# Autodesk Inventor assembly: MainAssembly
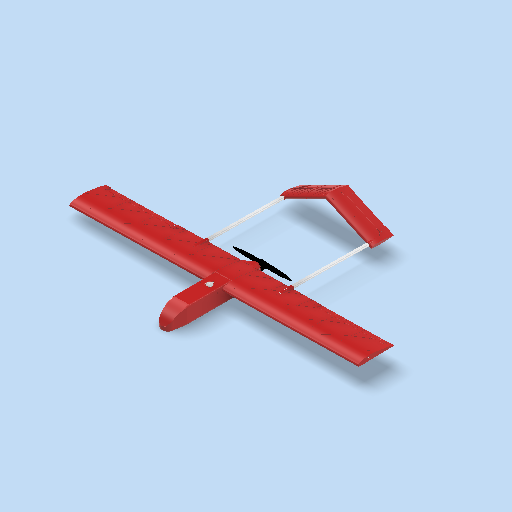
[picture p0: Inventor's stored thumbnail of the model, 512x512]
Saved by Autodesk Inventor 2026.1 (Build 301233000, 233)
## iProperties
Created: 2025-08-01
Part Number: MainAssembly
Document SubType Name: Assembly
Designer: Cupri
Author: Cupri
## Documents named in this file (29)
- C:\GitHub\SWIFT-UAV\System_development\Pelican\structural_model\v0.3.0\MainAssembly\MainAssembly.iam
- C:\GitHub\SWIFT-UAV\System_development\Pelican\structural_model\v0.3.0\Parts\WingParts\WingBox.ipt
- C:\GitHub\SWIFT-UAV\System_development\Pelican\structural_model\v0.3.0\Parts\WingParts\WingLeft_v0.1.ipt
- C:\GitHub\SWIFT-UAV\System_development\Pelican\structural_model\v0.3.0\Parts\Extrusion\20x20x1295ExtrudedAluminum.ipt
- C:\GitHub\SWIFT-UAV\System_development\Pelican\structural_model\v0.3.0\Parts\Extrusion\20x20x800ExtrudedAluminum.ipt
- C:\GitHub\SWIFT-UAV\System_development\Pelican\structural_model\v0.3.0\Parts\MotorHousing.ipt
- C:\GitHub\SWIFT-UAV\System_development\Pelican\structural_model\v0.3.0\Parts\Fueselage.ipt
- C:\GitHub\SWIFT-UAV\System_development\Pelican\structural_model\v0.3.0\Parts\FrontCover.ipt
- C:\GitHub\SWIFT-UAV\System_development\Pelican\structural_model\v0.3.0\Parts\AlerionLeft.ipt
- C:\GitHub\SWIFT-UAV\System_development\Pelican\structural_model\v0.3.0\Parts\Extrusion\20x20x1295ExtrudedAluminum_MIR.ipt
- C:\GitHub\SWIFT-UAV\System_development\Pelican\structural_model\v0.3.0\Parts\WingParts\WingLeft_v0.1_MIR1.ipt
- C:\GitHub\SWIFT-UAV\System_development\Pelican\structural_model\v0.3.0\Parts\Extrusion\20x20x800ExtrudedAluminum_MIR2.ipt
- C:\GitHub\SWIFT-UAV\System_development\Pelican\structural_model\v0.3.0\Parts\Vtail.ipt
- C:\GitHub\SWIFT-UAV\System_development\Pelican\structural_model\v0.3.0\Parts\Vtail_MIR.ipt
- C:\GitHub\SWIFT-UAV\System_development\Pelican\structural_model\v0.3.0\Parts\AlerionLeft_MIR1.ipt
- C:\GitHub\SWIFT-UAV\System_development\Pelican\structural_model\v0.3.0\Parts\Extrusion\20x20x785ExtrudedAluminum.ipt
- C:\GitHub\SWIFT-UAV\System_development\Pelican\structural_model\v0.3.0\Parts\Mount v2.ipt
- C:\GitHub\SWIFT-UAV\System_development\Pelican\structural_model\v0.3.0\Parts\kst-ds215mg-servo-1.snapshot.4\KST_DS215MG\KST_DS215MG\KST_DS215MG.ipt
- C:\GitHub\SWIFT-UAV\System_development\Pelican\structural_model\v0.3.0\Parts\WingParts\servo cap.ipt
- C:\GitHub\SWIFT-UAV\System_development\Pelican\structural_model\v0.3.0\Parts\WingParts\servo cap_MIR.ipt
- C:\GitHub\SWIFT-UAV\System_development\Pelican\structural_model\v0.3.0\Parts\Tail.ipt
- C:\GitHub\SWIFT-UAV\System_development\Pelican\structural_model\v0.3.0\Parts\WingParts\Wing servo cap.ipt
- C:\GitHub\SWIFT-UAV\System_development\Pelican\structural_model\v0.3.0\Parts\WingParts\Wing servo cap_MIR1.ipt
- C:\GitHub\SWIFT-UAV\System_development\Pelican\structural_model\v0.3.0\Parts\WingParts\servoarm.ipt
- C:\GitHub\SWIFT-UAV\System_development\Pelican\structural_model\v0.3.0\Parts\X7215\X7215\X7215.ipt
- C:\GitHub\SWIFT-UAV\System_development\Pelican\structural_model\v0.3.0\Parts\NutRetainer.ipt
- C:\GitHub\SWIFT-UAV\System_development\Pelican\structural_model\v0.3.0\Parts\Prop.ipt
- C:\GitHub\SWIFT-UAV\System_development\Pelican\structural_model\v0.3.0\Avionics\Pitot_tube.iam
- C:\GitHub\SWIFT-UAV\System_development\Pelican\structural_model\v0.3.0\Avionics\GPS Holybro.iam
## Components (31 placed, 28 different names)
1. Fueselage:1 — Mate:1, Flush:1, Flush:7, Mate:7, Mate:23, Mate:27, Mate:28, Mate:30, Mate:31, Mate:32, Flush:20, Flush:21, Mate:56, Mate:59, Mate:60, Mate:61, Mate:62
2. WingBox:1 — Mate:1, Mate:3, Angle:1, Flush:7
3. FrontCover:1 — Flush:1
4. 20x20x1295ExtrudedAluminum:1 — Mate:4, Mate:9
5. WingLeft_v0.1:1 — Mate:5, Angle:2, Mate:7, Mate:52, Flush:19, Insert:4
6. 20x20x800ExtrudedAluminum:1 — Mate:9, Flush:12, Mate:51, Mate:52
7. MotorHousing:1 — Flush:21, Mate:56, Mate:57, Mate:58
8. 20x20x1295ExtrudedAluminum_MIR:1 — Mate:16, Mate:19
9. WingLeft_v0.1_MIR1:1 — Mate:18, Insert:2
10. 20x20x800ExtrudedAluminum_MIR2:1 — Mate:19, Mate:49
11. Vtail:1 — Insert:3
12. Vtail_MIR:1 — Mate:44, Mate:45, Flush:18
13. AlerionLeft:1 — Insert:4
14. AlerionLeft_MIR1:1 — Insert:2
15. 20x20x785ExtrudedAluminum:1 — Mate:29, Mate:30, Mate:31, Mate:32
16. Mount v2:1 — Mate:25, Angle:6, Mate:27, Mate:28, Mate:29
17. KST_DS215MG:1
18. KST_DS215MG:2 — Mate:53
19. servo cap:1
20. servo cap_MIR:1
21. Tail:1 — Mate:34, Mate:38, Mate:39, Mate:43, Angle:8, Mate:44, Mate:45, Mate:46, Angle:9, Mate:50, Mate:53, Insert:3
22. Wing servo cap:1 — Flush:19
23. Wing servo cap_MIR1:1
24. servoarm:1
25. servoarm:2
26. X7215:1 — Mate:57, Mate:58
27. NutRetainer:3 — Mate:59, Mate:60
28. NutRetainer:4 — Mate:61, Mate:62
29. Prop:1
30. Pitot_tube:1 [sub-assembly]
31. GPS Holybro:1 [sub-assembly]
## Relationships (54: Mate 39, Flush 7, Angle 5, Insert 3)
- Mate:1: Fueselage:1 ↔ WingBox:1
- Flush:1: Fueselage:1 ↔ FrontCover:1
- Mate:3: WingBox:1
- Angle:1 (0 deg): WingBox:1
- Mate:4: 20x20x1295ExtrudedAluminum:1
- Mate:5: WingLeft_v0.1:1
- Angle:2 (0 deg): WingLeft_v0.1:1
- Flush:7: Fueselage:1 ↔ WingBox:1
- Mate:6
- Mate:7: Fueselage:1 ↔ WingLeft_v0.1:1
- Mate:9: 20x20x1295ExtrudedAluminum:1 ↔ 20x20x800ExtrudedAluminum:1
- Mate:15
- Mate:16: 20x20x1295ExtrudedAluminum_MIR:1
- Mate:17
- Mate:18: WingLeft_v0.1_MIR1:1
- Mate:19: 20x20x1295ExtrudedAluminum_MIR:1 ↔ 20x20x800ExtrudedAluminum_MIR2:1
- Flush:12 (-100 mm): 20x20x800ExtrudedAluminum:1
- Mate:23: Fueselage:1
- Mate:25: Mount v2:1
- Angle:6 (0 deg): Mount v2:1
- Mate:27 (0.25 mm): Fueselage:1 ↔ Mount v2:1
- Mate:28 (23 mm): Fueselage:1 ↔ Mount v2:1
- Mate:29 (0.5 mm): 20x20x785ExtrudedAluminum:1 ↔ Mount v2:1
- Mate:30: Fueselage:1 ↔ 20x20x785ExtrudedAluminum:1
- Mate:31: Fueselage:1 ↔ 20x20x785ExtrudedAluminum:1
- Mate:32: Fueselage:1 ↔ 20x20x785ExtrudedAluminum:1
- Mate:34: Tail:1
- Mate:38: Tail:1
- Mate:39: Tail:1
- Mate:43: Tail:1
- Angle:8 (0 deg): Tail:1
- Mate:44: Vtail_MIR:1 ↔ Tail:1
- Mate:45: Vtail_MIR:1 ↔ Tail:1
- Mate:46: Tail:1
- Angle:9 (0 deg): Tail:1
- Flush:18: Vtail_MIR:1
- Mate:49: 20x20x800ExtrudedAluminum_MIR2:1
- Mate:50: Tail:1
- Mate:51: 20x20x800ExtrudedAluminum:1
- Mate:52: WingLeft_v0.1:1 ↔ 20x20x800ExtrudedAluminum:1
- Mate:53 (0.25 mm): KST_DS215MG:2 ↔ Tail:1
- Flush:19: WingLeft_v0.1:1 ↔ Wing servo cap:1
- Flush:20: Fueselage:1
- Flush:21: Fueselage:1 ↔ MotorHousing:1
- Mate:56: Fueselage:1 ↔ MotorHousing:1
- Mate:57: MotorHousing:1 ↔ X7215:1
- Mate:58: MotorHousing:1 ↔ X7215:1
- Mate:59: Fueselage:1 ↔ NutRetainer:3
- Mate:60: Fueselage:1 ↔ NutRetainer:3
- Mate:61: Fueselage:1 ↔ NutRetainer:4
- Mate:62: Fueselage:1 ↔ NutRetainer:4
- Insert:2 (8 mm): WingLeft_v0.1_MIR1:1 ↔ AlerionLeft_MIR1:1
- Insert:3: Vtail:1 ↔ Tail:1
- Insert:4 (8 mm): WingLeft_v0.1:1 ↔ AlerionLeft:1
